# Autodesk Inventor assembly: Door Assembly revII
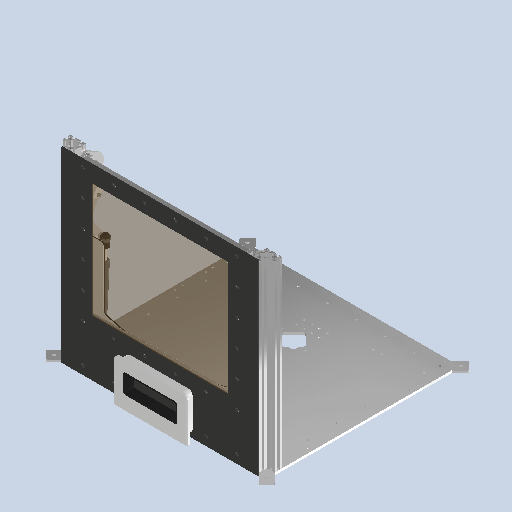
[picture p0: Inventor's stored thumbnail of the model, 512x512]
Saved by Autodesk Inventor 2024 (Build 280153000, 153)
## iProperties
Created: 2024-08-28
Part Number: Door Assembly revII
Document SubType Name: Assembly
Designer: Ishaan
Author: Ishaan
## Documents named in this file (33)
- E:\Projects\Axiom--IDEX-3D-Printer\CAD\06 - Door\Door Assembly revII.iam
- E:\Projects\Axiom--IDEX-3D-Printer\CAD\06 - Door\Door Aluminum Bars.ipt
- E:\Projects\Axiom--IDEX-3D-Printer\CAD\06 - Door\Door Lower Parallel Bar.ipt
- E:\Projects\Axiom--IDEX-3D-Printer\CAD\06 - Door\Door Upper Parallel Bar.ipt
- E:\Projects\Axiom--IDEX-3D-Printer\CAD\00 - COTS Components\F685ZZ.ipt
- E:\Projects\Axiom--IDEX-3D-Printer\CAD\06 - Door\Door Bar Bearing Spacer.ipt
- E:\Projects\Axiom--IDEX-3D-Printer\CAD\06 - Door\Door Bar Bearing Door Mounting Spacer.ipt
- E:\Projects\Axiom--IDEX-3D-Printer\CAD\06 - Door\Door Bar Bearing Frame Mounting Spacer.ipt
- E:\Projects\Axiom--IDEX-3D-Printer\CAD\00 - COTS Components\Hardware\SHCSM5x20.ipt
- E:\Projects\Axiom--IDEX-3D-Printer\CAD\00 - COTS Components\Hardware\M5 T SLOT NUT.ipt
- E:\Projects\Axiom--IDEX-3D-Printer\CAD\00 - COTS Components\Hardware\SHCSM5x16.ipt
- E:\Projects\Axiom--IDEX-3D-Printer\CAD\02 - Frame\Printer Base Plate RevII.ipt
- E:\Projects\Axiom--IDEX-3D-Printer\CAD\00 - COTS Components\2020 Door Runners\HFSC5-2020-425.ipt
- E:\Projects\Axiom--IDEX-3D-Printer\CAD\00 - COTS Components\2020 Door Bar Extrusion\HFSC5-2020-443.ipt
- E:\Projects\Axiom--IDEX-3D-Printer\CAD\06 - Door\Door Bar Brace Mount.ipt
- E:\Projects\Axiom--IDEX-3D-Printer\CAD\00 - COTS Components\Hardware\SHCSM5x25.ipt
- E:\Projects\Axiom--IDEX-3D-Printer\CAD\00 - COTS Components\Hardware\M5 LOCKNUT.ipt
- E:\Projects\Axiom--IDEX-3D-Printer\CAD\06 - Door\Door Stiffening Gusset.ipt
- E:\Projects\Axiom--IDEX-3D-Printer\CAD\00 - COTS Components\4040 Vertical L Extrusions\HFS5-404020-475-SC.ipt
- E:\Projects\Axiom--IDEX-3D-Printer\CAD\00 - COTS Components\Hardware\SHCSM5x8.ipt
- E:\Projects\Axiom--IDEX-3D-Printer\CAD\00 - COTS Components\Gas Strut Hardware\Gas Strut Ball Stud.ipt
- E:\Projects\Axiom--IDEX-3D-Printer\CAD\06 - Door\Gas Strut Lower Plate.ipt
- E:\Projects\Axiom--IDEX-3D-Printer\CAD\00 - COTS Components\Gas Strut Hardware\strut_assem\strut_assem_LH.iam
- E:\Projects\Axiom--IDEX-3D-Printer\CAD\00 - COTS Components\Gas Strut Hardware\strut_assem\strut_assem_UH.iam
- E:\Projects\Axiom--IDEX-3D-Printer\CAD\00 - COTS Components\Hardware\SHCSM5x12.ipt
- E:\Projects\Axiom--IDEX-3D-Printer\CAD\06 - Door\Door Stop.ipt
- E:\Projects\Axiom--IDEX-3D-Printer\CAD\06 - Door\Door Stop Bumper.ipt
- E:\Projects\Axiom--IDEX-3D-Printer\CAD\06 - Door\Door Bar Front Panel Mount.ipt
- E:\Projects\Axiom--IDEX-3D-Printer\CAD\00 - COTS Components\Hardware\M5 Heat Set Insert.ipt
- E:\Projects\Axiom--IDEX-3D-Printer\CAD\06 - Door\Door Panel R2.ipt
- E:\Projects\Axiom--IDEX-3D-Printer\CAD\00 - COTS Components\Hardware\FSCM5x8.ipt
- E:\Projects\Axiom--IDEX-3D-Printer\CAD\06 - Door\Door Window.ipt
- E:\Projects\Axiom--IDEX-3D-Printer\CAD\06 - Door\Door Handle.ipt
## Components (189 placed, 32 different names)
1. Door Aluminum Bars:1 — Insert:52, Insert:53, Insert:54, Insert:57, Angle:10, Insert:59, Angle:11, Insert:90, Insert:91, Insert:92, Insert:129, Insert:130, Insert:131
2. HFSC5-2020-425:1 — Insert:58, Insert:59, Angle:11
3. HFSC5-2020-425:2 — Insert:54, Insert:55, Angle:9
4. HFSC5-2020-425:3 — Insert:56, Insert:57, Angle:10
5. Door Aluminum Bars:2 — Insert:50, Insert:51, Insert:55, Angle:9, Insert:56, Insert:58, Insert:87, Insert:88, Insert:89, Insert:126, Insert:127, Insert:128
6. Printer Base Plate RevII:1 — Mate:11, Mate:15, Mate:18
7. HFS5-404020-475-SC:1 — DOOR_ANGLE, Mate:17, Mate:19
8. HFS5-404020-475-SC:2 — Mate:14, Mate:16
9. Door Lower Parallel Bar:1 — Insert:12, Insert:14, Insert:19, Insert:21, DOOR_ANGLE, Insert:63, Insert:64, Insert:66, Insert:67, Insert:71, Insert:93, Insert:105, Angle:18, Insert:118, Insert:119
10. Door Upper Parallel Bar:1 — Insert:1, Insert:3, Insert:7, Insert:9
11. Door Bar Bearing Spacer:1 — Insert:20
12. Door Bar Bearing Spacer:2 — Insert:13
13. Door Bar Bearing Door Mounting Spacer:1 — Insert:22, Insert:52
14. Door Lower Parallel Bar:2 — Insert:35, Insert:37, Insert:40, Insert:42, Insert:62, Insert:73, Insert:74, Insert:78, Insert:79, Insert:86, Insert:104, Angle:20, Insert:120, Insert:121
15. Door Bar Bearing Spacer:3 — Insert:36
16. Door Bar Bearing Spacer:4 — Insert:41
17. Door Bar Bearing Door Mounting Spacer:2 — Insert:39, Insert:50
18. Door Bar Bearing Frame Mounting Spacer:1 — Insert:16, Insert:17, Angle:2
19. Door Bar Bearing Frame Mounting Spacer:2 — Insert:43, Insert:44, Angle:4
20. Door Upper Parallel Bar:2 — Insert:24, Insert:26, Insert:29, Insert:31
21. Door Bar Bearing Spacer:5 — Insert:8
22. Door Bar Bearing Spacer:6 — Insert:2
23. Door Bar Bearing Spacer:7 — Insert:25
24. Door Bar Bearing Spacer:8 — Insert:30
25. Door Bar Bearing Door Mounting Spacer:3 — Insert:10, Insert:53
26. Door Bar Bearing Door Mounting Spacer:4 — Insert:27, Insert:51
27. Door Bar Bearing Frame Mounting Spacer:3 — Insert:33, Insert:34, Angle:3
28. Door Bar Bearing Frame Mounting Spacer:4 — Insert:4, Angle:1, Insert:18
29. HFSC5-2020-443:2 — Insert:62, Insert:63, Mate:13
30. Door Bar Brace Mount:1 — Insert:64, Insert:66, Insert:67, Insert:71, Insert:82, Insert:83, Insert:85, Angle:14, Insert:94, Mate:26
31. Door Bar Brace Mount:2 — Insert:73, Insert:74, Insert:78, Insert:79, Insert:80, Insert:81, Insert:84, Angle:15, Insert:96
32. Door Stiffening Gusset:1 — Insert:94, Mate:13, Insert:98, Insert:100, Insert:103, Angle:17
33. Door Stiffening Gusset:2 — Insert:96, Insert:99, Insert:101, Insert:102, Angle:16
34. Gas Strut Ball Stud:1 — Insert:104, Mate:24
35. Gas Strut Ball Stud:2 — Insert:105, Mate:20
36. Gas Strut Lower Plate:1 — Mate:17, Mate:18, Mate:19, Insert:109, Insert:110, Insert:111, Insert:114, Insert:115, Angle:22, Angle:23
37. Gas Strut Lower Plate:2 — Mate:14, Mate:15, Mate:16, Insert:108, Insert:112, Insert:113, Insert:116, Insert:117, Angle:24, Angle:25
38. Gas Strut Ball Stud:3 — Insert:109, Mate:21
39. Gas Strut Ball Stud:4 — Insert:108, Mate:23
40. strut_assem_LH:1 [sub-assembly] — Mate:21, Mate:22, Angle:19
41. strut_assem_UH:1 [sub-assembly] — Mate:20, Mate:22, Angle:18, Angle:19
42. strut_assem_LH:2 [sub-assembly] — Mate:23, Mate:25, Angle:21
43. strut_assem_UH:2 [sub-assembly] — Mate:24, Mate:25, Angle:20, Angle:21
44. Door Stop:1 — Insert:118, Insert:119, Insert:122, Insert:123, Mate:28, Angle:26, Mate:29
45. Door Stop:2 — Insert:120, Insert:121, Insert:124, Insert:125, Mate:30, Angle:27, Mate:31
46. Door Stop Bumper:1 — Mate:28, Angle:26, Mate:29
47. Door Stop Bumper:2 — Mate:30, Angle:27, Mate:31
48. Door Bar Front Panel Mount:1 — Insert:129, Insert:130, Insert:131, Insert:136, Insert:138, Insert:142
49. Door Bar Front Panel Mount:2 — Insert:126, Insert:127, Insert:128, Insert:132, Insert:137, Insert:143
50. Door Panel R2:1 — Insert:141, Insert:142, Insert:143, Mate:32, Mate:33, Mate:34, Insert:144, Angle:28, Insert:145, Angle:29, Insert:146, Angle:30, Insert:148, Insert:149, Insert:152
51. Door Window:1 — Mate:32, Mate:33, Mate:34
52. Door Handle:1 — Insert:148, Insert:149, Insert:150, Insert:151, Angle:31
53. SHCSM5x8:10 — Insert:122
54. SHCSM5x8:11 — Insert:123
55. SHCSM5x8:12 — Insert:124
56. SHCSM5x8:13 — Insert:125
57. SHCSM5x12:1 — Insert:110
58. SHCSM5x12:2 — Insert:111
59. SHCSM5x12:3 — Insert:112
60. SHCSM5x12:4 — Insert:113
61. M5 T SLOT NUT:15 — Insert:114, Angle:23
62. M5 T SLOT NUT:16 — Insert:115, Angle:22
63. M5 T SLOT NUT:17 — Insert:116, Angle:24
64. M5 T SLOT NUT:18 — Insert:117, Angle:25
65. SHCSM5x16:5 — Insert:86
66. SHCSM5x16:6 — Insert:87
67. SHCSM5x16:7 — Insert:88
68. SHCSM5x16:8 — Insert:89
69. SHCSM5x16:9 — Insert:90
70. SHCSM5x16:10 — Insert:91
71. SHCSM5x16:11 — Insert:92
72. SHCSM5x16:12 — Insert:93
73. SHCSM5x16:1 — Insert:11
74. SHCSM5x16:2 — Insert:23
75. SHCSM5x16:3 — Insert:28
76. SHCSM5x16:4 — Insert:38
77. SHCSM5x20:1 — Insert:32, Mate:5, Mate:6, Mate:11
78. SHCSM5x20:2 — Insert:45, Mate:5, Mate:8
79. SHCSM5x20:3 — Insert:5, Mate:6
80. SHCSM5x20:4 — Insert:15, Mate:8
81. M5 T SLOT NUT:1 — Insert:34, Angle:3
82. M5 T SLOT NUT:2 — Insert:44, Angle:4
83. M5 T SLOT NUT:3 — Insert:17, Angle:2
84. M5 T SLOT NUT:4 — Angle:1, Insert:18
85. F685ZZ:5 — Insert:35, Insert:36, Insert:38
86. F685ZZ:6 — Insert:42, Insert:43
87. F685ZZ:7 — Insert:37, Insert:39
88. F685ZZ:8 — Insert:40, Insert:41, Insert:45
89. F685ZZ:1 — Insert:19, Insert:20, Insert:22
90. F685ZZ:2 — Insert:12, Insert:13, Insert:15
91. F685ZZ:3 — Insert:21, Insert:23
92. F685ZZ:4 — Insert:14, Insert:16
93. F685ZZ:13 — Insert:24, Insert:25, Insert:28
94. F685ZZ:14 — Insert:29, Insert:30, Insert:33
95. F685ZZ:15 — Insert:26, Insert:27
96. F685ZZ:16 — Insert:31, Insert:32
97. F685ZZ:9 — Insert:9, Insert:10
98. F685ZZ:10 — Insert:1, Insert:2, Insert:5
99. F685ZZ:11 — Insert:7, Insert:8, Insert:11
100. F685ZZ:12 — Insert:3, Insert:4
101. SHCSM5x16:19 — Insert:150
102. SHCSM5x16:20
103. SHCSM5x16:21
104. M5 LOCKNUT:7 — Insert:151, Angle:31
105. M5 LOCKNUT:8
106. M5 LOCKNUT:9
107. SHCSM5x20:11 — Insert:152
108. SHCSM5x20:12
109. SHCSM5x20:13
110. FSCM5x8:1 — Insert:141
111. FSCM5x8:2
112. FSCM5x8:3
113. FSCM5x8:4
114. FSCM5x8:5
115. FSCM5x8:6
116. FSCM5x8:7
117. FSCM5x8:8
118. FSCM5x8:9
119. FSCM5x8:10
120. FSCM5x8:11
121. FSCM5x8:12
122. FSCM5x8:13
123. FSCM5x8:14
124. FSCM5x8:15
125. FSCM5x8:16
126. FSCM5x8:17
127. FSCM5x8:18
128. FSCM5x8:19
129. FSCM5x8:20
130. FSCM5x8:21
131. FSCM5x8:22
132. FSCM5x8:23
133. FSCM5x8:24
134. SHCSM5x20:6 — Insert:138
135. SHCSM5x20:7
136. SHCSM5x20:8
137. SHCSM5x20:5 — Insert:137
138. SHCSM5x20:9
139. SHCSM5x20:10
140. M5 Heat Set Insert:7 — Insert:136
141. M5 Heat Set Insert:8
142. M5 Heat Set Insert:9
143. M5 Heat Set Insert:10
144. M5 Heat Set Insert:6 — Insert:132
145. M5 Heat Set Insert:11
146. M5 Heat Set Insert:12
147. M5 Heat Set Insert:13
148. M5 T SLOT NUT:19 — Insert:144, Angle:28
149. M5 T SLOT NUT:20
150. M5 T SLOT NUT:21
151. M5 T SLOT NUT:22
152. M5 T SLOT NUT:23
153. M5 T SLOT NUT:24
154. M5 T SLOT NUT:25 — Insert:145, Angle:29
155. M5 T SLOT NUT:26
156. M5 T SLOT NUT:27
157. M5 T SLOT NUT:28
158. M5 T SLOT NUT:29 — Insert:146, Angle:30
159. M5 T SLOT NUT:30
160. M5 T SLOT NUT:31
161. M5 T SLOT NUT:32
162. M5 T SLOT NUT:5 — Insert:102, Angle:16
163. M5 T SLOT NUT:6
164. M5 T SLOT NUT:7
165. M5 T SLOT NUT:10 — Insert:103, Angle:17
166. M5 T SLOT NUT:11
167. M5 T SLOT NUT:12
168. SHCSM5x8:1 — Insert:100
169. SHCSM5x8:2
170. SHCSM5x8:8
171. SHCSM5x8:6 — Insert:101
172. SHCSM5x8:7
173. SHCSM5x8:9
174. SHCSM5x16:13 — Insert:98
175. SHCSM5x16:14 — Mate:26
176. SHCSM5x16:17 — Insert:99
177. SHCSM5x16:18 — Mate:27
178. SHCSM5x25:9 — Insert:82
179. SHCSM5x25:10 — Insert:83
180. SHCSM5x25:11
181. SHCSM5x25:12
182. M5 LOCKNUT:1 — Insert:84, Angle:15
183. M5 LOCKNUT:3 — Mate:27
184. M5 LOCKNUT:2 — Insert:85, Angle:14
185. M5 LOCKNUT:6
186. SHCSM5x25:1 — Insert:81
187. SHCSM5x25:2 — Insert:80
188. SHCSM5x25:3
189. SHCSM5x25:4
## Component patterns: (3 elements, first: SHCSM5x16:19), (3 elements, first: M5 LOCKNUT:7), (3 elements, first: SHCSM5x20:11), (24 elements, first: FSCM5x8:1), (3 elements, first: SHCSM5x20:6), (3 elements, first: SHCSM5x20:5), (4 elements, first: M5 Heat Set Insert:7), (4 elements, first: M5 Heat Set Insert:6), (6 elements, first: M5 T SLOT NUT:19), (4 elements, first: M5 T SLOT NUT:25), (4 elements, first: M5 T SLOT NUT:29), (3 elements, first: M5 T SLOT NUT:5), (3 elements, first: M5 T SLOT NUT:10), (3 elements, first: SHCSM5x8:1), (3 elements, first: SHCSM5x8:6), (2 elements, first: SHCSM5x16:13), (2 elements, first: SHCSM5x16:17), (2 elements, first: SHCSM5x25:9 + SHCSM5x25:10), (2 elements, first: M5 LOCKNUT:1), (2 elements, first: M5 LOCKNUT:2), (2 elements, first: SHCSM5x25:1 + SHCSM5x25:2)
## Relationships (194: Insert 131, Mate 32, Angle 31)
- Insert:1: Door Upper Parallel Bar:1 ↔ F685ZZ:10
- Insert:2 (0.1 mm): Door Bar Bearing Spacer:6 ↔ F685ZZ:10
- Insert:3: Door Upper Parallel Bar:1 ↔ F685ZZ:12
- Insert:4: Door Bar Bearing Frame Mounting Spacer:4 ↔ F685ZZ:12
- Insert:5: SHCSM5x20:3 ↔ F685ZZ:10
- Angle:1 (0 deg): Door Bar Bearing Frame Mounting Spacer:4 ↔ M5 T SLOT NUT:4
- Insert:7: Door Upper Parallel Bar:1 ↔ F685ZZ:11
- Insert:8 (0.1 mm): Door Bar Bearing Spacer:5 ↔ F685ZZ:11
- Insert:9: Door Upper Parallel Bar:1 ↔ F685ZZ:9
- Insert:10: Door Bar Bearing Door Mounting Spacer:3 ↔ F685ZZ:9
- Insert:11: SHCSM5x16:1 ↔ F685ZZ:11
- Insert:12: Door Lower Parallel Bar:1 ↔ F685ZZ:2
- Insert:13 (0.1 mm): Door Bar Bearing Spacer:2 ↔ F685ZZ:2
- Insert:14: Door Lower Parallel Bar:1 ↔ F685ZZ:4
- Insert:15: SHCSM5x20:4 ↔ F685ZZ:2
- Insert:16: Door Bar Bearing Frame Mounting Spacer:1 ↔ F685ZZ:4
- Insert:17 (2 mm): Door Bar Bearing Frame Mounting Spacer:1 ↔ M5 T SLOT NUT:3
- Angle:2 (0 deg): Door Bar Bearing Frame Mounting Spacer:1 ↔ M5 T SLOT NUT:3
- Insert:18 (2 mm): Door Bar Bearing Frame Mounting Spacer:4 ↔ M5 T SLOT NUT:4
- Insert:19: Door Lower Parallel Bar:1 ↔ F685ZZ:1
- Insert:20: Door Bar Bearing Spacer:1 ↔ F685ZZ:1
- Insert:21: Door Lower Parallel Bar:1 ↔ F685ZZ:3
- Insert:22: Door Bar Bearing Door Mounting Spacer:1 ↔ F685ZZ:1
- Insert:23: SHCSM5x16:2 ↔ F685ZZ:3
- Insert:24: Door Upper Parallel Bar:2 ↔ F685ZZ:13
- Insert:25: Door Bar Bearing Spacer:7 ↔ F685ZZ:13
- Insert:26: Door Upper Parallel Bar:2 ↔ F685ZZ:15
- Insert:27: Door Bar Bearing Door Mounting Spacer:4 ↔ F685ZZ:15
- Insert:28: SHCSM5x16:3 ↔ F685ZZ:13
- Insert:29: Door Upper Parallel Bar:2 ↔ F685ZZ:14
- Insert:30: Door Bar Bearing Spacer:8 ↔ F685ZZ:14
- Insert:31: Door Upper Parallel Bar:2 ↔ F685ZZ:16
- Insert:32: SHCSM5x20:1 ↔ F685ZZ:16
- Insert:33: Door Bar Bearing Frame Mounting Spacer:3 ↔ F685ZZ:14
- Insert:34 (2 mm): Door Bar Bearing Frame Mounting Spacer:3 ↔ M5 T SLOT NUT:1
- Angle:3 (0 deg): Door Bar Bearing Frame Mounting Spacer:3 ↔ M5 T SLOT NUT:1
- Insert:35: Door Lower Parallel Bar:2 ↔ F685ZZ:5
- Insert:36: Door Bar Bearing Spacer:3 ↔ F685ZZ:5
- Insert:37: Door Lower Parallel Bar:2 ↔ F685ZZ:7
- Insert:38: SHCSM5x16:4 ↔ F685ZZ:5
- Insert:39: Door Bar Bearing Door Mounting Spacer:2 ↔ F685ZZ:7
- Insert:40: Door Lower Parallel Bar:2 ↔ F685ZZ:8
- Insert:41: Door Bar Bearing Spacer:4 ↔ F685ZZ:8
- Insert:42: Door Lower Parallel Bar:2 ↔ F685ZZ:6
- Insert:43: Door Bar Bearing Frame Mounting Spacer:2 ↔ F685ZZ:6
- Insert:44 (2 mm): Door Bar Bearing Frame Mounting Spacer:2 ↔ M5 T SLOT NUT:2
- Angle:4 (0 deg): Door Bar Bearing Frame Mounting Spacer:2 ↔ M5 T SLOT NUT:2
- Insert:45: SHCSM5x20:2 ↔ F685ZZ:8
- [Insert]: Printer Base Plate RevII:1 ↔ HFS5-404020-475-SC:1
- [Insert]: Printer Base Plate RevII:1 ↔ HFS5-404020-475-SC:1
- [Insert]: Printer Base Plate RevII:1 ↔ HFS5-404020-475-SC:2
- [Insert]: Printer Base Plate RevII:1 ↔ HFS5-404020-475-SC:2
- [Mate]: HFS5-404020-475-SC:2 ↔ Door Bar Bearing Frame Mounting Spacer:3
- [Mate] (-10 mm): HFS5-404020-475-SC:2 ↔ SHCSM5x20:1
- [Mate]: HFS5-404020-475-SC:2 ↔ Door Bar Bearing Frame Mounting Spacer:2
- [Mate] (-10 mm): HFS5-404020-475-SC:2 ↔ SHCSM5x20:2
- Insert:50: Door Aluminum Bars:2 ↔ Door Bar Bearing Door Mounting Spacer:2
- Insert:51: Door Aluminum Bars:2 ↔ Door Bar Bearing Door Mounting Spacer:4
- Mate:5 (147 mm): SHCSM5x20:1 ↔ SHCSM5x20:2
- [Angle] (0 deg): HFS5-404020-475-SC:2 ↔ Door Bar Bearing Frame Mounting Spacer:3
- [Angle] (0 deg): HFS5-404020-475-SC:2 ↔ Door Bar Bearing Frame Mounting Spacer:2
- Mate:6: SHCSM5x20:1 ↔ SHCSM5x20:3
- [Mate]: HFS5-404020-475-SC:1 ↔ Door Bar Bearing Frame Mounting Spacer:4
- [Angle] (0 deg): HFS5-404020-475-SC:1 ↔ Door Bar Bearing Frame Mounting Spacer:4
- Mate:8: SHCSM5x20:2 ↔ SHCSM5x20:4
- [Mate]: HFS5-404020-475-SC:1 ↔ Door Bar Bearing Frame Mounting Spacer:1
- [Angle] (0 deg): HFS5-404020-475-SC:1 ↔ Door Bar Bearing Frame Mounting Spacer:1
- Insert:52: Door Aluminum Bars:1 ↔ Door Bar Bearing Door Mounting Spacer:1
- Insert:53: Door Aluminum Bars:1 ↔ Door Bar Bearing Door Mounting Spacer:3
- Insert:54: Door Aluminum Bars:1 ↔ HFSC5-2020-425:2
- Insert:55: HFSC5-2020-425:2 ↔ Door Aluminum Bars:2
- Angle:9 (0 deg): HFSC5-2020-425:2 ↔ Door Aluminum Bars:2
- Insert:56: HFSC5-2020-425:3 ↔ Door Aluminum Bars:2
- Insert:57: Door Aluminum Bars:1 ↔ HFSC5-2020-425:3
- Angle:10 (0 deg): Door Aluminum Bars:1 ↔ HFSC5-2020-425:3
- Insert:58: HFSC5-2020-425:1 ↔ Door Aluminum Bars:2
- Insert:59: Door Aluminum Bars:1 ↔ HFSC5-2020-425:1
- Angle:11 (0 deg): Door Aluminum Bars:1 ↔ HFSC5-2020-425:1
- [Angle] (0 deg): HFSC5-2020-425:1 ↔ HFS5-404020-475-SC:2
- Mate:11 (460 mm): Printer Base Plate RevII:1 ↔ SHCSM5x20:1
- DOOR_ANGLE [Angle] (30 deg): HFS5-404020-475-SC:1 ↔ Door Lower Parallel Bar:1
- Insert:62: Door Lower Parallel Bar:2 ↔ HFSC5-2020-443:2
- Insert:63: Door Lower Parallel Bar:1 ↔ HFSC5-2020-443:2
- Insert:64: Door Lower Parallel Bar:1 ↔ Door Bar Brace Mount:1
- Insert:66: Door Lower Parallel Bar:1 ↔ Door Bar Brace Mount:1
- Insert:67: Door Lower Parallel Bar:1 ↔ Door Bar Brace Mount:1
- Insert:71: Door Lower Parallel Bar:1 ↔ Door Bar Brace Mount:1
- Insert:73: Door Lower Parallel Bar:2 ↔ Door Bar Brace Mount:2
- Insert:74: Door Lower Parallel Bar:2 ↔ Door Bar Brace Mount:2
- Insert:78: Door Lower Parallel Bar:2 ↔ Door Bar Brace Mount:2
- Insert:79: Door Lower Parallel Bar:2 ↔ Door Bar Brace Mount:2
- Insert:80: Door Bar Brace Mount:2 ↔ SHCSM5x25:2
- Insert:81: Door Bar Brace Mount:2 ↔ SHCSM5x25:1
- Insert:82: Door Bar Brace Mount:1 ↔ SHCSM5x25:9
- Insert:83: Door Bar Brace Mount:1 ↔ SHCSM5x25:10
- Insert:84: Door Bar Brace Mount:2 ↔ M5 LOCKNUT:1
- Insert:85: Door Bar Brace Mount:1 ↔ M5 LOCKNUT:2
- Angle:14 (0 deg): Door Bar Brace Mount:1 ↔ M5 LOCKNUT:2
- Angle:15 (0 deg): Door Bar Brace Mount:2 ↔ M5 LOCKNUT:1
- Insert:86: Door Lower Parallel Bar:2 ↔ SHCSM5x16:5
- Insert:87: Door Aluminum Bars:2 ↔ SHCSM5x16:6
- Insert:88: Door Aluminum Bars:2 ↔ SHCSM5x16:7
- Insert:89: Door Aluminum Bars:2 ↔ SHCSM5x16:8
- Insert:90: Door Aluminum Bars:1 ↔ SHCSM5x16:9
- Insert:91: Door Aluminum Bars:1 ↔ SHCSM5x16:10
- Insert:92: Door Aluminum Bars:1 ↔ SHCSM5x16:11
- Insert:93: Door Lower Parallel Bar:1 ↔ SHCSM5x16:12
- Insert:94 (0.25 mm): Door Bar Brace Mount:1 ↔ Door Stiffening Gusset:1
- Mate:13: HFSC5-2020-443:2 ↔ Door Stiffening Gusset:1
- Insert:96 (0.25 mm): Door Bar Brace Mount:2 ↔ Door Stiffening Gusset:2
- Insert:98: Door Stiffening Gusset:1 ↔ SHCSM5x16:13
- Insert:99: Door Stiffening Gusset:2 ↔ SHCSM5x16:17
- Insert:100: Door Stiffening Gusset:1 ↔ SHCSM5x8:1
- Insert:101: Door Stiffening Gusset:2 ↔ SHCSM5x8:6
- Insert:102 (2 mm): Door Stiffening Gusset:2 ↔ M5 T SLOT NUT:5
- Angle:16 (0 deg): Door Stiffening Gusset:2 ↔ M5 T SLOT NUT:5
- Insert:103 (2 mm): Door Stiffening Gusset:1 ↔ M5 T SLOT NUT:10
- Angle:17 (0 deg): Door Stiffening Gusset:1 ↔ M5 T SLOT NUT:10
- Insert:104: Door Lower Parallel Bar:2 ↔ Gas Strut Ball Stud:1
- Insert:105: Door Lower Parallel Bar:1 ↔ Gas Strut Ball Stud:2
- Mate:14: HFS5-404020-475-SC:2 ↔ Gas Strut Lower Plate:2
- Mate:15: Printer Base Plate RevII:1 ↔ Gas Strut Lower Plate:2
- Mate:16 (-10 mm): HFS5-404020-475-SC:2 ↔ Gas Strut Lower Plate:2
- Mate:17: HFS5-404020-475-SC:1 ↔ Gas Strut Lower Plate:1
- Mate:18: Printer Base Plate RevII:1 ↔ Gas Strut Lower Plate:1
- Mate:19 (-10 mm): HFS5-404020-475-SC:1 ↔ Gas Strut Lower Plate:1
- Insert:108: Gas Strut Lower Plate:2 ↔ Gas Strut Ball Stud:4
- Insert:109: Gas Strut Lower Plate:1 ↔ Gas Strut Ball Stud:3
- Mate:20: Gas Strut Ball Stud:2 ↔ strut_assem_UH:1
- Mate:21: Gas Strut Ball Stud:3 ↔ strut_assem_LH:1
- Mate:22: strut_assem_LH:1 ↔ strut_assem_UH:1
- Angle:18 (175 deg): Door Lower Parallel Bar:1 ↔ strut_assem_UH:1
- Angle:19 (0 deg): strut_assem_LH:1 ↔ strut_assem_UH:1
- Mate:23: Gas Strut Ball Stud:4 ↔ strut_assem_LH:2
- Mate:24: Gas Strut Ball Stud:1 ↔ strut_assem_UH:2
- Mate:25: strut_assem_LH:2 ↔ strut_assem_UH:2
- Angle:20 (175 deg): Door Lower Parallel Bar:2 ↔ strut_assem_UH:2
- Angle:21 (0 deg): strut_assem_LH:2 ↔ strut_assem_UH:2
- Insert:110: Gas Strut Lower Plate:1 ↔ SHCSM5x12:1
- Insert:111: Gas Strut Lower Plate:1 ↔ SHCSM5x12:2
- Insert:112: Gas Strut Lower Plate:2 ↔ SHCSM5x12:3
- Insert:113: Gas Strut Lower Plate:2 ↔ SHCSM5x12:4
- Insert:114 (2 mm): Gas Strut Lower Plate:1 ↔ M5 T SLOT NUT:15
- Insert:115 (2 mm): Gas Strut Lower Plate:1 ↔ M5 T SLOT NUT:16
- Angle:22 (0 deg): Gas Strut Lower Plate:1 ↔ M5 T SLOT NUT:16
- Angle:23 (0 deg): Gas Strut Lower Plate:1 ↔ M5 T SLOT NUT:15
- Insert:116 (2 mm): Gas Strut Lower Plate:2 ↔ M5 T SLOT NUT:17
- Insert:117 (2 mm): Gas Strut Lower Plate:2 ↔ M5 T SLOT NUT:18
- Angle:24 (0 deg): Gas Strut Lower Plate:2 ↔ M5 T SLOT NUT:17
- Angle:25 (0 deg): Gas Strut Lower Plate:2 ↔ M5 T SLOT NUT:18
- Mate:26: Door Bar Brace Mount:1 ↔ SHCSM5x16:14
- Mate:27: SHCSM5x16:18 ↔ M5 LOCKNUT:3
- Insert:118: Door Lower Parallel Bar:1 ↔ Door Stop:1
- Insert:119: Door Lower Parallel Bar:1 ↔ Door Stop:1
- Insert:120: Door Lower Parallel Bar:2 ↔ Door Stop:2
- Insert:121: Door Lower Parallel Bar:2 ↔ Door Stop:2
- Insert:122: Door Stop:1 ↔ SHCSM5x8:10
- Insert:123: Door Stop:1 ↔ SHCSM5x8:11
- Insert:124: Door Stop:2 ↔ SHCSM5x8:12
- Insert:125: Door Stop:2 ↔ SHCSM5x8:13
- Mate:28: Door Stop:1 ↔ Door Stop Bumper:1
- Angle:26 (180 deg): Door Stop:1 ↔ Door Stop Bumper:1
- Mate:29 (0.2 mm): Door Stop:1 ↔ Door Stop Bumper:1
- Mate:30: Door Stop:2 ↔ Door Stop Bumper:2
- Angle:27 (180 deg): Door Stop:2 ↔ Door Stop Bumper:2
- Mate:31 (0.2 mm): Door Stop:2 ↔ Door Stop Bumper:2
- Insert:126: Door Aluminum Bars:2 ↔ Door Bar Front Panel Mount:2
- Insert:127: Door Aluminum Bars:2 ↔ Door Bar Front Panel Mount:2
- Insert:128: Door Aluminum Bars:2 ↔ Door Bar Front Panel Mount:2
- Insert:129: Door Aluminum Bars:1 ↔ Door Bar Front Panel Mount:1
- Insert:130: Door Aluminum Bars:1 ↔ Door Bar Front Panel Mount:1
- Insert:131: Door Aluminum Bars:1 ↔ Door Bar Front Panel Mount:1
- Insert:132: Door Bar Front Panel Mount:2 ↔ M5 Heat Set Insert:6
- Insert:136: Door Bar Front Panel Mount:1 ↔ M5 Heat Set Insert:7
- Insert:137: Door Bar Front Panel Mount:2 ↔ SHCSM5x20:5
- Insert:138: Door Bar Front Panel Mount:1 ↔ SHCSM5x20:6
- Insert:141: Door Panel R2:1 ↔ FSCM5x8:1
- Insert:142: Door Bar Front Panel Mount:1 ↔ Door Panel R2:1
- Insert:143: Door Bar Front Panel Mount:2 ↔ Door Panel R2:1
- Mate:32: Door Panel R2:1 ↔ Door Window:1
- Mate:33 (0.5 mm): Door Panel R2:1 ↔ Door Window:1
- Mate:34 (0.5 mm): Door Panel R2:1 ↔ Door Window:1
- Insert:144 (2 mm): Door Panel R2:1 ↔ M5 T SLOT NUT:19
- Angle:28 (0 deg): Door Panel R2:1 ↔ M5 T SLOT NUT:19
- Insert:145 (2 mm): Door Panel R2:1 ↔ M5 T SLOT NUT:25
- Angle:29 (0 deg): Door Panel R2:1 ↔ M5 T SLOT NUT:25
- Insert:146 (2 mm): Door Panel R2:1 ↔ M5 T SLOT NUT:29
- Angle:30 (0 deg): Door Panel R2:1 ↔ M5 T SLOT NUT:29
- Insert:148: Door Panel R2:1 ↔ Door Handle:1
- Insert:149: Door Panel R2:1 ↔ Door Handle:1
- Insert:150: Door Handle:1 ↔ SHCSM5x16:19
- Insert:151: Door Handle:1 ↔ M5 LOCKNUT:7
- Angle:31 (0 deg): Door Handle:1 ↔ M5 LOCKNUT:7
- Insert:152: Door Panel R2:1 ↔ SHCSM5x20:11
